# Autodesk Inventor assembly: Assemblage_général
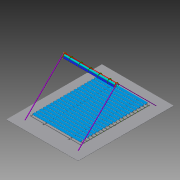
[picture p0: Inventor's stored thumbnail of the model, 180x180]
Saved by Autodesk Inventor 2015 SP1 (Build 190203100, 203)
## iProperties
Created: 2015-04-17
Part Number: Assemblage_général
Document SubType Name: Assembly
Designer: Cyril
Author: Cyril
## Documents named in this file (6)
- C:\Users\Cyril\Documents\OSE FR\Concentrateur solaire\Inventor\Assemblage_général_N-S.iam
- C:\Users\Cyril\Documents\OSE FR\Concentrateur solaire\Inventor\Assemblage_cadre-miroir.iam
- C:\Users\Cyril\Documents\OSE FR\Concentrateur solaire\Inventor\Poutre.ipt
- C:\Users\Cyril\Documents\OSE FR\Concentrateur solaire\Inventor\Sol.ipt
- C:\Users\Cyril\Documents\OSE FR\Concentrateur solaire\Inventor\Pied.ipt
- C:\Users\Cyril\Documents\OSE FR\Concentrateur solaire\Inventor\Absorbeur\Assemblage absorbeur N-S.iam
## Components (7 placed, 5 different names)
1. Sol:1 — Mate:10, Mate:11, Flush:8, Mate:13, Mate:15, Mate:18, Flush:9, Mate:19
2. Poutre:2 — Insert:6, Angle:1, Mate:13, Insert:7, Insert:8, Insert:9, Insert:10
3. Pied:1 — Insert:6, Angle:1
4. Assemblage_cadre-miroir:1 [sub-assembly] — Mate:18, Insert:9, Insert:10, Flush:9, Insert:11
5. Assemblage_cadre-miroir:2 [sub-assembly] — Insert:7, Insert:8, Insert:12
6. Assemblage absorbeur N-S:1 [sub-assembly] — Mate:15, Mate:19
7. Poutre:3 — Insert:11, Insert:12
## Relationships (16: Insert 7, Mate 6, Flush 2, Angle 1)
- Insert:6: Poutre:2 ↔ Pied:1
- Angle:1 (180 deg): Poutre:2 ↔ Pied:1
- Mate:10: Sol:1
- Mate:11: Sol:1
- Flush:8: Sol:1
- Mate:13: Sol:1 ↔ Poutre:2
- Mate:15: Sol:1 ↔ Assemblage absorbeur N-S:1
- Mate:18: Sol:1 ↔ Assemblage_cadre-miroir:1
- Insert:7: Poutre:2 ↔ Assemblage_cadre-miroir:2
- Insert:8: Poutre:2 ↔ Assemblage_cadre-miroir:2
- Insert:9: Poutre:2 ↔ Assemblage_cadre-miroir:1
- Insert:10: Poutre:2 ↔ Assemblage_cadre-miroir:1
- Flush:9: Sol:1 ↔ Assemblage_cadre-miroir:1
- Mate:19: Sol:1 ↔ Assemblage absorbeur N-S:1
- Insert:11: Assemblage_cadre-miroir:1 ↔ Poutre:3
- Insert:12: Assemblage_cadre-miroir:2 ↔ Poutre:3
